# Autodesk Inventor assembly: xMotor
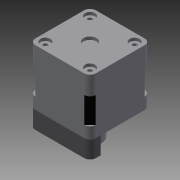
[picture p0: Inventor's stored thumbnail of the model, 180x180]
Saved by Autodesk Inventor 2013 (Build 170138000, 138)
## iProperties
Created: 2015-01-14
Part Number: xMotor
Document SubType Name: Assembly
Designer: dzban
Author: dzban
## Documents named in this file (4)
- D:\PIRX\Artisan\OPENSOURCE\SmallPieces\xMotor.iam
- D:\PIRX\Artisan\OPENSOURCE\SmallPieces\xMotorSpacer.ipt
- D:\PIRX\Artisan\OPENSOURCE\StockComponents\NEMA17Stepper.ipt
- D:\PIRX\Artisan\OPENSOURCE\StockComponents\gt2_20_pulley.ipt
## Components (4 placed, 3 different names)
1. xMotorSpacer:1 — Insert:1, Insert:2, Insert:3, Insert:4
2. xMotorSpacer:2 — Insert:3, Insert:4
3. NEMA17Stepper:1 — Insert:1, Insert:2, Insert:5
4. gt2_20_pulley:1 — Insert:5
## Relationships (5: Insert 5)
- Insert:1: xMotorSpacer:1 ↔ NEMA17Stepper:1
- Insert:2: xMotorSpacer:1 ↔ NEMA17Stepper:1
- Insert:3: xMotorSpacer:1 ↔ xMotorSpacer:2
- Insert:4: xMotorSpacer:1 ↔ xMotorSpacer:2
- Insert:5 (1 mm): NEMA17Stepper:1 ↔ gt2_20_pulley:1
